# Autodesk Inventor assembly: S2x1
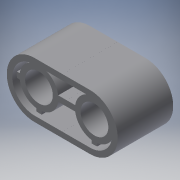
[picture p0: Inventor's stored thumbnail of the model, 180x180]
Saved by Autodesk Inventor 2019.3 (Build 233278000, 278)
## iProperties
Created: 2019-01-31
Part Number: S2x1
Document SubType Name: Assembly
Designer: Varga Daniel
Author: Varga Daniel
## Documents named in this file (3)
- C:\!_Dani\!_cloud\OneDrive\!_munka\Revolution\RevvyDemoKit\Structural parts\Beams\Straight Beams\S2+x1\S2x1.iam
- C:\!_Dani\!_cloud\OneDrive\!_munka\Revolution\RevvyDemoKit\Structural parts\Beams\beam_single_end_part.ipt
- C:\!_Dani\!_cloud\OneDrive\!_munka\Revolution\RevvyDemoKit\Structural parts\Beams\Straight Beams\S2+x1.iam
## Components (2 placed, 1 different names)
1. beam_single_end_part:1 — Flush:1, Flush:2, Mate:1
2. beam_single_end_part:2 — Flush:1, Flush:2, Mate:1
## Relationships (3: Flush 2, Mate 1)
- Flush:1: beam_single_end_part:1 ↔ beam_single_end_part:2
- Flush:2: beam_single_end_part:1 ↔ beam_single_end_part:2
- Mate:1: beam_single_end_part:1 ↔ beam_single_end_part:2
